# Autodesk Inventor assembly: TinyFan_Extrusion_Explosion
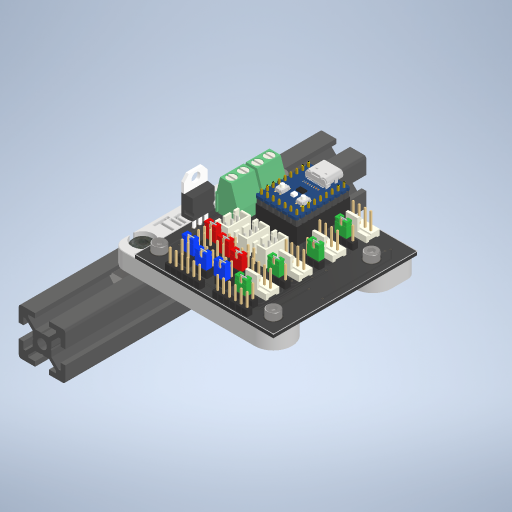
[picture p0: Inventor's stored thumbnail of the model, 512x512]
Saved by Autodesk Inventor 2023.1 (Build 271208000, 208)
## iProperties
Created: 2022-09-15
Part Number: TinyFan_Extrusion_Explosion
Document SubType Name: Assembly
Designer: Rama
Author: Rama
## Documents named in this file (8)
- C:\Users\Rama\Desktop\GitHub\TinyFan\CAD\SRC\TinyFan_Extrusion_Assembled.iam
- C:\Users\Rama\Desktop\GitHub\TinyFan\CAD\SRC\TinyFan_Extrusion_1pc_90.ipt
- C:\Users\Rama\Desktop\GitHub\TrashInventor\M3 Threaded Insert.ipt
- C:\Users\Rama\Documents\Inventor\Content Center Files\R2023\de-DE\DIN 912\DIN 912 - M3 x 0,5 x 8 x 6,75.ipt
- C:\Users\Rama\Documents\Inventor\Content Center Files\R2023\de-DE\ISO 7380-1\ISO 7380-1 - M5 x 8.ipt
- C:\Users\Rama\Desktop\GitHub\TrashInventor\HFSB5-2020-130.ipt
- C:\Users\Rama\Desktop\GitHub\TrashInventor\SHNTP5-5.ipt
- C:\Users\Rama\Desktop\Neuer Ordner\tiny-fan-traces.iam
## Components (15 placed, 7 different names)
1. tiny-fan-traces:1 [sub-assembly]
2. TinyFan_Extrusion_1pc_90:1 — Passend:3, Passend:4, Passend:5, Passend:6, Passend:11, Passend:12, Fluchtend:10, Fluchtend:11, Passend:17, Passend:20
3. M3 Threaded Insert:1 — Passend:3, Fluchtend:3, Fluchtend:11
4. M3 Threaded Insert:2 — Passend:6, Fluchtend:1
5. M3 Threaded Insert:3 — Passend:5, Fluchtend:1, Fluchtend:2
6. M3 Threaded Insert:4 — Passend:4, Fluchtend:2, Fluchtend:3
7. DIN 912 - ersetzt durch DIN EN ISO 4762 M3 x 8:1 — Fluchtend:5, Fluchtend:6
8. DIN 912 - ersetzt durch DIN EN ISO 4762 M3 x 8:2 — Fluchtend:6
9. DIN 912 - ersetzt durch DIN EN ISO 4762 M3 x 8:3 — Fluchtend:4
10. DIN 912 - ersetzt durch DIN EN ISO 4762 M3 x 8:4 — Fluchtend:4, Fluchtend:5
11. ISO 7380-1 M5 x 8:1 — Passend:11, Fluchtend:7, Passend:13, Passend:17
12. ISO 7380-1 M5 x 8:2 — Passend:12, Fluchtend:7, Passend:14
13. HFSB5-2020-130:1 — Passend:15, Winkel:1, Fluchtend:10, Passend:16, Passend:20
14. SHNTP5-5:1 — Passend:13, Fluchtend:8, Fluchtend:9, Passend:16
15. SHNTP5-5:2 — Passend:14, Fluchtend:8, Fluchtend:9, Passend:15, Winkel:1
## Relationships (32: Mate 20, Flush 11, Angle 1)
- [Mate]: tiny-fan-traces:1 ↔ TinyFan_Extrusion_1pc_90:1
- [Mate]: tiny-fan-traces:1 ↔ TinyFan_Extrusion_1pc_90:1
- Passend:3 [Mate]: TinyFan_Extrusion_1pc_90:1 ↔ M3 Threaded Insert:1
- Passend:4 [Mate]: TinyFan_Extrusion_1pc_90:1 ↔ M3 Threaded Insert:4
- Passend:5 [Mate]: TinyFan_Extrusion_1pc_90:1 ↔ M3 Threaded Insert:3
- Passend:6 [Mate]: TinyFan_Extrusion_1pc_90:1 ↔ M3 Threaded Insert:2
- Fluchtend:1 [Flush]: M3 Threaded Insert:2 ↔ M3 Threaded Insert:3
- Fluchtend:2 [Flush]: M3 Threaded Insert:3 ↔ M3 Threaded Insert:4
- Fluchtend:3 [Flush]: M3 Threaded Insert:1 ↔ M3 Threaded Insert:4
- [Mate]: tiny-fan-traces:1 ↔ DIN 912 - ersetzt durch DIN EN ISO 4762 M3 x 8:4
- [Mate]: tiny-fan-traces:1 ↔ DIN 912 - ersetzt durch DIN EN ISO 4762 M3 x 8:2
- [Mate]: tiny-fan-traces:1 ↔ DIN 912 - ersetzt durch DIN EN ISO 4762 M3 x 8:1
- [Mate]: tiny-fan-traces:1 ↔ DIN 912 - ersetzt durch DIN EN ISO 4762 M3 x 8:3
- Fluchtend:4 [Flush]: DIN 912 - ersetzt durch DIN EN ISO 4762 M3 x 8:3 ↔ DIN 912 - ersetzt durch DIN EN ISO 4762 M3 x 8:4
- Fluchtend:5 [Flush]: DIN 912 - ersetzt durch DIN EN ISO 4762 M3 x 8:1 ↔ DIN 912 - ersetzt durch DIN EN ISO 4762 M3 x 8:4
- Fluchtend:6 [Flush]: DIN 912 - ersetzt durch DIN EN ISO 4762 M3 x 8:1 ↔ DIN 912 - ersetzt durch DIN EN ISO 4762 M3 x 8:2
- Passend:11 [Mate]: TinyFan_Extrusion_1pc_90:1 ↔ ISO 7380-1 M5 x 8:1
- Passend:12 [Mate]: TinyFan_Extrusion_1pc_90:1 ↔ ISO 7380-1 M5 x 8:2
- Fluchtend:7 [Flush]: ISO 7380-1 M5 x 8:1 ↔ ISO 7380-1 M5 x 8:2
- Passend:13 [Mate]: ISO 7380-1 M5 x 8:1 ↔ SHNTP5-5:1
- Passend:14 [Mate]: ISO 7380-1 M5 x 8:2 ↔ SHNTP5-5:2
- Fluchtend:8 [Flush]: SHNTP5-5:1 ↔ SHNTP5-5:2
- Fluchtend:9 [Flush]: SHNTP5-5:1 ↔ SHNTP5-5:2
- Passend:15 [Mate] (0.1 mm): HFSB5-2020-130:1 ↔ SHNTP5-5:2
- Winkel:1 [Angle] (0 deg): HFSB5-2020-130:1 ↔ SHNTP5-5:2
- Fluchtend:10 [Flush] (-35 mm): TinyFan_Extrusion_1pc_90:1 ↔ HFSB5-2020-130:1
- Passend:16 [Mate]: HFSB5-2020-130:1 ↔ SHNTP5-5:1
- Fluchtend:11 [Flush]: TinyFan_Extrusion_1pc_90:1 ↔ M3 Threaded Insert:1
- Passend:17 [Mate]: TinyFan_Extrusion_1pc_90:1 ↔ ISO 7380-1 M5 x 8:1
- [Mate]: tiny-fan-traces:1 ↔ DIN 912 - ersetzt durch DIN EN ISO 4762 M3 x 8:2
- [Mate]: tiny-fan-traces:1 ↔ TinyFan_Extrusion_1pc_90:1
- Passend:20 [Mate]: TinyFan_Extrusion_1pc_90:1 ↔ HFSB5-2020-130:1
